# Autodesk Inventor assembly: Assembly2
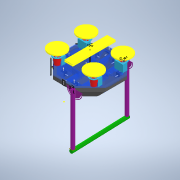
[picture p0: Inventor's stored thumbnail of the model, 180x180]
Saved by Autodesk Inventor 2020.2 (Build 242310000, 310)
## iProperties
Created: 2020-02-17
Part Number: Assembly2
Document SubType Name: Assembly
Designer: lenovo
Author: lenovo
## Documents named in this file (19)
- D:\BE II Year\eng exploration\notes\Assembly2.iam
- D:\BE II Year\eng exploration\notes\trail 2.ipt
- D:\BE II Year\eng exploration\notes\trail 3.1.ipt
- D:\BE II Year\eng exploration\notes\trail 8.ipt
- D:\BE II Year\eng exploration\notes\trail 4.ipt
- D:\BE II Year\eng exploration\notes\trail 7.ipt
- D:\BE II Year\eng exploration\notes\trail 6.1.ipt
- D:\BE II Year\eng exploration\notes\trail 5.ipt
- D:\BE II Year\eng exploration\notes\trail 10.ipt
- D:\BE II Year\eng exploration\notes\trail 11.ipt
- D:\BE II Year\eng exploration\notes\Assembly3.iam
- D:\BE II Year\eng exploration\notes\trail 13.ipt
- D:\BE II Year\eng exploration\notes\trail 14.ipt
- D:\BE II Year\eng exploration\notes\trail 12.ipt
- D:\BE II Year\eng exploration\notes\trail 9.ipt
- D:\BE II Year\eng exploration\notes\trail 15.ipt
- D:\BE II Year\eng exploration\notes\trail 16.ipt
- D:\BE II Year\eng exploration\notes\trail 17.ipt
- D:\BE II Year\eng exploration\notes\downloads\Files\LED_Complete.iam
## Components (64 placed, 18 different names)
1. trail 2:1 — Rotational:1, Rotational:2, Rotational:3, Rotational:4, Rotational:12, Rotational:13, Rotational:14, Rigid:3, Rigid:4, Rigid:5, Rigid:6, Rigid:7, Rigid:8, Rigid:9, Rigid:10, Rigid:11, Rotational:15
2. trail 3.1:2 — Rotational:1, Rotational:8
3. trail 3.1:3 — Rotational:2, Rotational:5
4. trail 3.1:4 — Rotational:3, Rotational:6
5. trail 3.1:5 — Rotational:4, Rotational:7
6. trail 8:1 — Rotational:6, Rotational:11
7. trail 8:2 — Rotational:7, Rotational:10
8. trail 8:3 — Rotational:5, Rigid:1
9. trail 8:4 — Rotational:8, Rotational:9
10. trail 4:1 — Rotational:9, Rigid:27
11. trail 4:2 — Rotational:10, Cylindrical:3
12. trail 4:3 — Rigid:1, Cylindrical:2
13. trail 4:4 — Rotational:11, Rigid:26
14. trail 7:1 — Rotational:12, Rigid:2, Flush:2
15. trail 6.1:1 — Rigid:2, Rotational:16, Rigid:12, Rotational:26, Rotational:27, Rotational:30, Rotational:31
16. trail 5:1 — Rotational:13
17. trail 5:2 — Rotational:14
18. trail 10:1 — Rotational:16, Rotational:17, Rigid:13
19. trail 11:1 — Rigid:4, Rotational:18, Rigid:16
20. trail 11:2 — Rigid:3, Rotational:20, Rigid:18
21. trail 11:3 — Rigid:11, Rigid:17, Rotational:19
22. trail 11:4 — Rigid:6, Rigid:24, Rigid:25
23. trail 11:5 — Rigid:5, Rigid:19, Rigid:20
24. trail 11:6 — Rigid:9, Rotational:23, Rotational:24
25. trail 11:7 — Rigid:8, Rotational:21, Rotational:22
26. trail 11:9 — Rigid:10, Rigid:23, Rotational:25
27. trail 11:10 — Rigid:7, Rigid:21, Rigid:22
28. trail 10:3 — Rotational:15, Rigid:14, Rigid:15
29. Assembly3:1 [sub-assembly] — Rigid:12, Rotational:26, Flush:1
30. trail 13:1 — Rotational:17
31. trail 13:2 — Rigid:13
32. trail 13:3 — Rigid:14
33. trail 13:4 — Rigid:15
34. trail 13:6 — Rigid:16
35. trail 13:7 — Rotational:19
36. trail 13:8 — Rigid:18
37. trail 13:9 — Rigid:20
38. trail 13:10 — Rigid:19
39. trail 13:11 — Rotational:20
40. trail 13:12 — Rigid:17
41. trail 13:13 — Rotational:18
42. trail 13:14 — Rigid:21
43. trail 13:15 — Rigid:22
44. trail 13:16 — Rotational:24
45. trail 13:17 — Rotational:23
46. trail 13:18 — Rotational:22
47. trail 13:19 — Rotational:21
48. trail 13:20 — Rigid:23
49. trail 13:21 — Rotational:25
50. trail 13:22 — Rigid:24
51. trail 13:23 — Rigid:25
52. trail 14:1 — Cylindrical:2
53. trail 14:2 — Rigid:26
54. trail 14:3 — Cylindrical:3
55. trail 14:4 — Rigid:27
56. trail 12:1 — Rotational:27, Rotational:28
57. trail 9:1 — Rotational:28
58. trail 15:1 — Flush:1
59. trail 16:1 — Flush:2
60. trail 17:2 — Rigid:28, Rotational:29
61. trail 13:24 — Rotational:29
62. trail 13:25 — Rigid:28
63. LED_Complete:1 [sub-assembly] — Rotational:30
64. LED_Complete:2 [sub-assembly] — Rotational:31
## Relationships (63: RevoluteJoint 31, WeldJoint 28, CylindricalJoint 2, Flush 2)
- Rotational:1 [RevoluteJoint] (10 mm): trail 2:1 ↔ trail 3.1:2
- Rotational:2 [RevoluteJoint] (10 mm): trail 2:1 ↔ trail 3.1:3
- Rotational:3 [RevoluteJoint] (10 mm): trail 2:1 ↔ trail 3.1:4
- Rotational:4 [RevoluteJoint] (-10 mm): trail 2:1 ↔ trail 3.1:5
- Rotational:5 [RevoluteJoint] (10 mm): trail 3.1:3 ↔ trail 8:3
- Rotational:6 [RevoluteJoint] (10 mm): trail 3.1:4 ↔ trail 8:1
- Rotational:7 [RevoluteJoint] (10 mm): trail 3.1:5 ↔ trail 8:2
- Rotational:8 [RevoluteJoint] (10 mm): trail 3.1:2 ↔ trail 8:4
- Rigid:1 [WeldJoint]: trail 8:3 ↔ trail 4:3
- Rotational:9 [RevoluteJoint]: trail 8:4 ↔ trail 4:1
- Rotational:10 [RevoluteJoint]: trail 8:2 ↔ trail 4:2
- Rotational:11 [RevoluteJoint]: trail 8:1 ↔ trail 4:4
- Rotational:12 [RevoluteJoint] (40 mm): trail 2:1 ↔ trail 7:1
- Rigid:2 [WeldJoint] (170 mm): trail 7:1 ↔ trail 6.1:1
- Rotational:13 [RevoluteJoint]: trail 2:1 ↔ trail 5:1
- Rotational:14 [RevoluteJoint]: trail 2:1 ↔ trail 5:2
- Rigid:3 [WeldJoint]: trail 2:1 ↔ trail 11:2
- Rigid:4 [WeldJoint]: trail 2:1 ↔ trail 11:1
- Rigid:5 [WeldJoint]: trail 2:1 ↔ trail 11:5
- Rigid:6 [WeldJoint]: trail 2:1 ↔ trail 11:4
- Rigid:7 [WeldJoint]: trail 2:1 ↔ trail 11:10
- Rigid:8 [WeldJoint]: trail 2:1 ↔ trail 11:7
- Rigid:9 [WeldJoint]: trail 2:1 ↔ trail 11:6
- Rigid:10 [WeldJoint]: trail 2:1 ↔ trail 11:9
- Rigid:11 [WeldJoint]: trail 2:1 ↔ trail 11:3
- Rotational:15 [RevoluteJoint]: trail 2:1 ↔ trail 10:3
- Rotational:16 [RevoluteJoint]: trail 6.1:1 ↔ trail 10:1
- Rigid:12 [WeldJoint]: trail 6.1:1 ↔ Assembly3:1
- Rotational:17 [RevoluteJoint]: trail 10:1 ↔ trail 13:1
- Rigid:13 [WeldJoint]: trail 10:1 ↔ trail 13:2
- Rigid:14 [WeldJoint]: trail 10:3 ↔ trail 13:3
- Rigid:15 [WeldJoint]: trail 10:3 ↔ trail 13:4
- Rotational:18 [RevoluteJoint]: trail 11:1 ↔ trail 13:13
- Rigid:16 [WeldJoint]: trail 11:1 ↔ trail 13:6
- Rigid:17 [WeldJoint]: trail 11:3 ↔ trail 13:12
- Rotational:19 [RevoluteJoint]: trail 11:3 ↔ trail 13:7
- Rotational:20 [RevoluteJoint]: trail 11:2 ↔ trail 13:11
- Rigid:18 [WeldJoint]: trail 11:2 ↔ trail 13:8
- Rigid:19 [WeldJoint]: trail 11:5 ↔ trail 13:10
- Rigid:20 [WeldJoint]: trail 11:5 ↔ trail 13:9
- Rigid:21 [WeldJoint]: trail 11:10 ↔ trail 13:14
- Rigid:22 [WeldJoint]: trail 11:10 ↔ trail 13:15
- Rotational:21 [RevoluteJoint]: trail 11:7 ↔ trail 13:19
- Rotational:22 [RevoluteJoint]: trail 11:7 ↔ trail 13:18
- Rotational:23 [RevoluteJoint]: trail 11:6 ↔ trail 13:17
- Rotational:24 [RevoluteJoint]: trail 11:6 ↔ trail 13:16
- Rigid:23 [WeldJoint]: trail 11:9 ↔ trail 13:20
- Rotational:25 [RevoluteJoint]: trail 11:9 ↔ trail 13:21
- Rigid:24 [WeldJoint]: trail 11:4 ↔ trail 13:22
- Rigid:25 [WeldJoint]: trail 11:4 ↔ trail 13:23
- Cylindrical:2: trail 4:3 ↔ trail 14:1
- Rigid:26 [WeldJoint] (-8 mm): trail 4:4 ↔ trail 14:2
- Cylindrical:3: trail 4:2 ↔ trail 14:3
- Rigid:27 [WeldJoint] (-8 mm): trail 4:1 ↔ trail 14:4
- Rotational:26 [RevoluteJoint] (2 mm): trail 6.1:1 ↔ Assembly3:1
- Rotational:27 [RevoluteJoint]: trail 6.1:1 ↔ trail 12:1
- Rotational:28 [RevoluteJoint]: trail 12:1 ↔ trail 9:1
- Flush:1: Assembly3:1 ↔ trail 15:1
- Flush:2: trail 7:1 ↔ trail 16:1
- Rigid:28 [WeldJoint]: trail 17:2 ↔ trail 13:25
- Rotational:29 [RevoluteJoint]: trail 17:2 ↔ trail 13:24
- Rotational:30 [RevoluteJoint]: trail 6.1:1 ↔ LED_Complete:1
- Rotational:31 [RevoluteJoint]: trail 6.1:1 ↔ LED_Complete:2
